# Autodesk Inventor assembly: ASY МОО 001 отстойник осветлитель
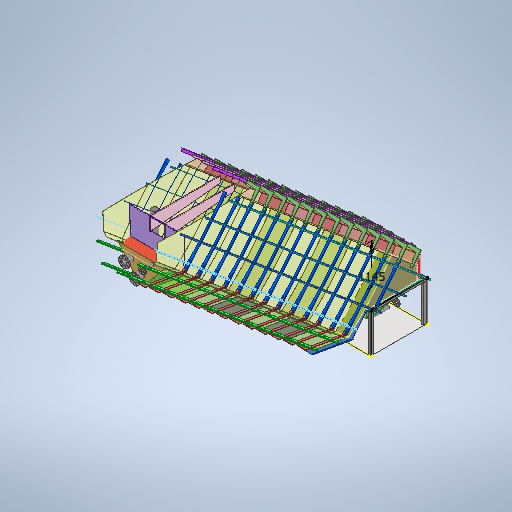
[picture p0: Inventor's stored thumbnail of the model, 512x512]
Saved by Autodesk Inventor 2025 (Build 290162010, 162A)
## iProperties
Created: 2024-04-28
Part Number: ASY МОО 001 отстойник осветлитель
Document SubType Name: Weldment
Designer: admin
Weld Material: Welded Aluminum-6061
Mass: 1.58517e+06 g
Surface Area: 1.48953e+06 cm^2
Volume: 226523 cm^3
Density: 6.99781 g/cm^3
Author: admin
## Documents named in this file (51)
- C:\Users\admin\YandexDisk-badmisterfox\домашниий пк\Inventor\Manturovo\Manturovo_Se-clar\ASY МОО 001 отстойник осветлитель.iam
- C:\Users\admin\YandexDisk-badmisterfox\домашниий пк\Inventor\Manturovo\Manturovo_Se-clar\MSC 033 sheet back basic.ipt
- C:\Users\admin\YandexDisk-badmisterfox\домашниий пк\Inventor\Manturovo\Manturovo_Se-clar\Пример емкости.ipt
- C:\Users\admin\YandexDisk-badmisterfox\домашниий пк\Inventor\Manturovo\Manturovo_Se-clar\MSC 041 sheet belly main.ipt
- C:\Users\admin\YandexDisk-badmisterfox\домашниий пк\Inventor\Manturovo\Manturovo_Se-clar\MSC 052 rib board.ipt
- C:\Users\admin\YandexDisk-badmisterfox\домашниий пк\Inventor\Manturovo\Manturovo_Se-clar\MSC 051 rib back.ipt
- C:\Users\admin\YandexDisk-badmisterfox\домашниий пк\Inventor\Manturovo\Manturovo_Se-clar\Рама основания\ASY MSC 090 base frame.iam
- C:\Users\admin\YandexDisk-badmisterfox\домашниий пк\Inventor\Manturovo\Manturovo_Se-clar\ASY MSC 080 roсket.iam
- C:\Users\admin\YandexDisk-badmisterfox\домашниий пк\Inventor\Manturovo\Manturovo_Se-clar\Content Center Files\en-US\ISO 5251 B 3D\ISO 5251 Bends 3D without straight ends(90 deg) DN80 2 2.ipt
- C:\Users\admin\YandexDisk-badmisterfox\домашниий пк\Inventor\Manturovo\Manturovo_Se-clar\Content Center Files\en-US\ISO 5251(1)\ISO 5251 Concentric reducers DN80 x DN65 3,2 3,2.ipt
- C:\Users\admin\YandexDisk-badmisterfox\домашниий пк\Inventor\Manturovo\Manturovo_Se-clar\ASY MSC 010 cone.iam
- C:\Users\admin\YandexDisk-badmisterfox\домашниий пк\Inventor\Manturovo\Manturovo_Se-clar\ракета\МОО 064 ракета труба.ipt
- C:\Users\admin\YandexDisk-badmisterfox\домашниий пк\Inventor\Manturovo\Manturovo_Se-clar\MSC 000 DIM settler-clarifier.ipt
- C:\Users\admin\YandexDisk-badmisterfox\домашниий пк\Inventor\Manturovo\Manturovo_Se-clar\MSC 031 sheet lowerback.ipt
- C:\Users\admin\YandexDisk-badmisterfox\домашниий пк\Inventor\Manturovo\Manturovo_Se-clar\Content Center Files\en-US\DIN EN 1092-1 01 - PN 25\DIN EN 1092-1 Plate Flange for Welding Type 01 - PN 25 80 x 88.9.ipt
- C:\Users\admin\YandexDisk-badmisterfox\домашниий пк\Inventor\Manturovo\Manturovo_Se-clar\MSC 024 sheet board main.ipt
- C:\Users\admin\YandexDisk-badmisterfox\домашниий пк\Inventor\Manturovo\Manturovo_Se-clar\MSC 032 sheet magic back-lowerback.ipt
- C:\Users\admin\YandexDisk-badmisterfox\домашниий пк\Inventor\Manturovo\Manturovo_Se-clar\MSC 021 sheet left board hip.ipt
- C:\Users\admin\YandexDisk-badmisterfox\домашниий пк\Inventor\Manturovo\Manturovo_Se-clar\MSC 022 sheet right board hip.ipt
- C:\Users\admin\YandexDisk-badmisterfox\домашниий пк\Inventor\Manturovo\Manturovo_Se-clar\MSC 034 sheet back-neck.ipt
- C:\Users\admin\YandexDisk-badmisterfox\домашниий пк\Inventor\Manturovo\Manturovo_Se-clar\MSC 042 sheet belly-neck.ipt
- C:\Users\admin\YandexDisk-badmisterfox\домашниий пк\Inventor\Manturovo\Manturovo_Se-clar\MSC 023 sheet board.ipt
- C:\Users\admin\YandexDisk-badmisterfox\домашниий пк\Inventor\Manturovo\Manturovo_Se-clar\конус\MSC 071 ridge 1.ipt
- C:\Users\admin\YandexDisk-badmisterfox\домашниий пк\Inventor\Manturovo\Manturovo_Se-clar\конус\MSC 073 ridge 3.ipt
- C:\Users\admin\YandexDisk-badmisterfox\домашниий пк\Inventor\Manturovo\Manturovo_Se-clar\конус\MSC 074 face 1.ipt
- C:\Users\admin\YandexDisk-badmisterfox\домашниий пк\Inventor\Manturovo\Manturovo_Se-clar\Content Center Files\en-US\ISO 5251 B 3D\ISO 5251 Bends 3D without straight ends(90 deg) DN150 11 11.ipt
- C:\Users\admin\YandexDisk-badmisterfox\домашниий пк\Inventor\Manturovo\Manturovo_Se-clar\Content Center Files\en-US\DIN EN 1092-1 01 - PN 25\DIN EN 1092-1 Plate Flange for Welding Type 01 - PN 25 150 x 168.3.ipt
- C:\Users\admin\YandexDisk-badmisterfox\домашниий пк\Inventor\Manturovo\Manturovo_Se-clar\МОО 061 труба верх 1.ipt
- C:\Users\admin\YandexDisk-badmisterfox\домашниий пк\Inventor\Manturovo\Manturovo_Se-clar\МОО 062 труба верх 2.ipt
- C:\Users\admin\YandexDisk-badmisterfox\домашниий пк\Inventor\Manturovo\Manturovo_Se-clar\МОО 063 труба верх 3.ipt
- C:\Users\admin\YandexDisk-badmisterfox\домашниий пк\Inventor\Manturovo\Manturovo_Se-clar\MSC 061 stringer back ^.ipt
- C:\Users\admin\YandexDisk-badmisterfox\домашниий пк\Inventor\Manturovo\Manturovo_Se-clar\MSC 063 stringer board #.ipt
- C:\Users\admin\YandexDisk-badmisterfox\домашниий пк\Inventor\Manturovo\Manturovo_Se-clar\MSC 062 stringer back ^^.ipt
- C:\Users\admin\YandexDisk-badmisterfox\домашниий пк\Inventor\Manturovo\Manturovo_Se-clar\MSC 064 stringer board ##.ipt
- C:\Users\admin\YandexDisk-badmisterfox\домашниий пк\Inventor\Manturovo\Manturovo_Se-clar\MSC 065 stringer board ###.ipt
- C:\Users\admin\YandexDisk-badmisterfox\домашниий пк\Inventor\Manturovo\Manturovo_Se-clar\MSC 066 stringer board ####.ipt
- C:\Users\admin\YandexDisk-badmisterfox\домашниий пк\Inventor\Manturovo\Manturovo_Se-clar\MSC 067 stringer board belly.ipt
- C:\Users\admin\YandexDisk-badmisterfox\домашниий пк\Inventor\Manturovo\Manturovo_Se-clar\MSC 053 rib belly.ipt
- C:\Users\admin\YandexDisk-badmisterfox\домашниий пк\Inventor\Manturovo\Manturovo_Se-clar\MSC 025 sheet board withers 1.ipt
- C:\Users\admin\YandexDisk-badmisterfox\домашниий пк\Inventor\Manturovo\Manturovo_Se-clar\MSC 027 sheet board face 1.ipt
- C:\Users\admin\YandexDisk-badmisterfox\домашниий пк\Inventor\Manturovo\Manturovo_Se-clar\Part1.ipt
- C:\Users\admin\YandexDisk-badmisterfox\домашниий пк\Inventor\Manturovo\Manturovo_Se-clar\стапель\ASY стапель.iam
- C:\Users\admin\YandexDisk-badmisterfox\домашниий пк\Inventor\Manturovo\Manturovo_Se-clar\DXF файлы\Шпангоуты+стрингеры\MSC 0101 sheet gills.ipt
- C:\Users\admin\YandexDisk-badmisterfox\домашниий пк\Inventor\Manturovo\Manturovo_Se-clar\MSC 026 sheet board withers 2.ipt
- C:\Users\admin\YandexDisk-badmisterfox\домашниий пк\Inventor\Manturovo\Manturovo_Se-clar\MSC 028 sheet board face 2.ipt
- C:\Users\admin\YandexDisk-badmisterfox\домашниий пк\Inventor\Manturovo\Manturovo_Se-clar\MSC 068 stringer lowerback.ipt
- C:\Users\admin\YandexDisk-badmisterfox\домашниий пк\Inventor\Manturovo\Manturovo_Se-clar\конус\MSC 072 ridge 2.ipt
- C:\Users\admin\YandexDisk-badmisterfox\домашниий пк\Inventor\Manturovo\Manturovo_Se-clar\MSC 075 face 2.ipt
- C:\Users\admin\YandexDisk-badmisterfox\домашниий пк\Inventor\Manturovo\Manturovo_Se-clar\MSC 076 face 3.ipt
- C:\Users\admin\YandexDisk-badmisterfox\домашниий пк\Inventor\Manturovo\Manturovo_Se-clar\MSC 077 face 4.ipt
- C:\Users\admin\YandexDisk-badmisterfox\домашниий пк\Inventor\Manturovo\Manturovo_Se-clar\MSC 052 rib board_CPY.ipt
## Components (226 placed, 57 different names)
1. Пример емкости.ipt:1 — Mate:1, Mate:2, Flush:2
2. MSC 000 DIM settler-clarifier.ipt:1
3. ASY MSC 090 base frame.iam:1 [sub-assembly] — Flush:19, Flush:21, Mate:82
4. MSC 033 sheet back basic.ipt:1 — Flush:3, Rigid:11, Rigid:12
5. MSC 041 sheet belly main.ipt:1 — Mate:9, Rigid:18, Rigid:40
6. ASY MSC 080 roсket.iam:1 [sub-assembly] — Flush:23, Rigid:10
7. ISO 5251 Bends 3D without straight ends(90 deg) DN80 2 2.ipt:1 — Rigid:2, Rigid:3
8. ISO 5251 Concentric reducers DN80 x DN65 3,2 3,2.ipt:1 — Rigid:2, Rigid:10, Mate:79
9. ASY MSC 010 cone.iam:1 [sub-assembly] — Flush:22, Mate:16, Flush:28, Mate:31, Mate:36, Mate:54, Mate:57, Mate:65, Mate:78, Tangent:11, Mate:79, Flush:79, Mate:82
10. МОО 064 ракета труба.ipt:1 — Rigid:3, Cylindrical:1
11. MSC 033 sheet back basic.ipt:2 — Rigid:11, Tangent:1, Tangent:3, Rigid:37
12. MSC 033 sheet back basic.ipt:3 — Flush:24, Rigid:12, Mate:19, Mate:22, Rigid:30, Mate:31, Flush:44, Tangent:8, Tangent:9
13. MSC 031 sheet lowerback.ipt:1 — Mate:15, Mate:16, Mate:19, Mate:22, Tangent:10, Tangent:11
14. DIN EN 1092-1 Plate Flange for Welding Type 01 - PN 25 80 x 88.9.ipt:1 — Flush:25, Flush:26, Mate:18, Cylindrical:1
15. MSC 024 sheet board main.ipt:1 — Flush:30, Tangent:1, Rigid:35, Mate:37
16. MSC 041 sheet belly main.ipt:2 — Rigid:18, Rigid:53
17. MSC 032 sheet magic back-lowerback.ipt:1 — Mate:24, Rigid:30, Flush:42, Tangent:6, Flush:43, Tangent:7
18. MSC 021 sheet left board hip.ipt:1 — Flush:41, Flush:42, Tangent:6, Mate:78
19. MSC 022 sheet right board hip.ipt:1 — Mate:30, Flush:43, Tangent:7
20. MSC 024 sheet board main.ipt:2 — Rigid:35, Rigid:36
21. MSC 024 sheet board main.ipt:3 — Rigid:36, Rigid:49
22. MSC 033 sheet back basic.ipt:4 — Rigid:37, Rigid:38
23. MSC 033 sheet back basic.ipt:5 — Rigid:38, Rigid:39
24. MSC 034 sheet back-neck.ipt:1 — Rigid:39
25. MSC 041 sheet belly main.ipt:3 — Rigid:40, Rigid:47
26. MSC 042 sheet belly-neck.ipt:1 — Rigid:48, Mate:70, Mate:71
27. MSC 041 sheet belly main.ipt:4 — Rigid:45, Rigid:47
28. MSC 041 sheet belly main.ipt:5 — Rigid:45, Rigid:48
29. MSC 024 sheet board main.ipt:4 — Rigid:49, Rigid:50
30. MSC 024 sheet board main.ipt:5 — Rigid:50, Rigid:113
31. MSC 023 sheet board.ipt:1 — Mate:36, Flush:47, Tangent:8, Mate:37, Mate:55
32. MSC 071 ridge 1.ipt:1 — Mate:50, Flush:57, Mate:68, Flush:81
33. MSC 074 face 1.ipt:1 — Rigid:156, Rigid:157, Mate:70, Flush:62, Mate:71, Rigid:159, Mate:80
34. MSC 041 sheet belly main.ipt:6 — Mate:54, Mate:55, Rigid:53
35. DIN EN 1092-1 Plate Flange for Welding Type 01 - PN 25 80 x 88.9.ipt:2 — Rigid:62
36. MSC 073 ridge 3.ipt:1 — Flush:56, Flush:57, Mate:68, Mate:77, Flush:78, Mate:81, Flush:80
37. DIN EN 1092-1 Plate Flange for Welding Type 01 - PN 25 150 x 168.3.ipt:1 — Rigid:158
38. МОО 061 труба верх 1.ipt:1 — Rigid:158, Rigid:59, Rigid:159
39. ISO 5251 Bends 3D without straight ends(90 deg) DN150 11 11.ipt:1 — Rigid:59, Rotational:2
40. МОО 062 труба верх 2.ipt:1 — Rigid:132, Rigid:156
41. DIN EN 1092-1 Plate Flange for Welding Type 01 - PN 25 150 x 168.3.ipt:2 — Rigid:132
42. МОО 063 труба верх 3.ipt:1 — Rigid:62, Rigid:157
43. MSC 024 sheet board main.ipt:6 — Rigid:134
44. MSC 024 sheet board main.ipt:7
45. MSC 024 sheet board main.ipt:8
46. MSC 024 sheet board main.ipt:9
47. MSC 024 sheet board main.ipt:10 — Rigid:67
48. MSC 023 sheet board.ipt:2 — Rigid:67, Mate:57, Mate:58, Tangent:9
49. MSC 052 rib board.ipt:1 — Rigid:74, Rigid:161, Rigid:162, Rigid:163, Rigid:164
50. MSC 051 rib back.ipt:1 — Rigid:25, Rigid:74, Rigid:91, Rigid:93, Rigid:139
51. MSC 066 stringer board ####.ipt:1 — Rigid:143, Rigid:162
52. MSC 065 stringer board ###.ipt:1 — Rigid:142, Rigid:163
53. MSC 064 stringer board ##.ipt:1 — Rigid:141, Rigid:164
54. MSC 063 stringer board #.ipt:1 — Rigid:140
55. MSC 062 stringer back ^^.ipt:1 — Rigid:93, Rigid:155
56. MSC 061 stringer back ^.ipt:2 — Rigid:91, Rigid:153
57. MSC 061 stringer back ^.ipt:1 — Rigid:90, Rigid:152
58. MSC 025 sheet board withers 1.ipt:1 — Rigid:113, Rigid:114
59. MSC 027 sheet board face 1.ipt:1 — Rigid:114, Flush:56, Mate:69, Flush:60, Mate:75
60. Part1.ipt:1
61. MSC 051 rib back.ipt:2 — Rigid:116, Rigid:130, Rigid:131, Rigid:169
62. MSC 051 rib back.ipt:3 — Rigid:116, Rigid:165
63. MSC 051 rib back.ipt:4 — Rigid:131
64. MSC 051 rib back.ipt:5 — Mate:62, Flush:53
65. MSC 062 stringer back ^^.ipt:2 — Rigid:92, Mate:66, Rigid:154
66. MSC 066 stringer board ####.ipt:2 — Rigid:125, Rigid:151
67. MSC 063 stringer board #.ipt:2 — Rigid:148
68. MSC 064 stringer board ##.ipt:2 — Rigid:149, Rigid:167
69. MSC 065 stringer board ###.ipt:2 — Rigid:150, Rigid:166
70. MSC 052 rib board.ipt:3 — Rigid:72, Flush:51, Flush:52, Rigid:125, Mate:61, Rigid:166, Rigid:167, Rigid:168
71. MSC 051 rib back.ipt:6 — Flush:12, Tangent:3, Rigid:25, Flush:44, Rigid:72, Rigid:90, Rigid:92, Rigid:130
72. ASY стапель.iam:1 [sub-assembly] — Mate:62, Flush:53, Mate:63
73. MSC 053 rib belly.ipt:2 — Rigid:110, Flush:51, Flush:52, Rigid:126, Mate:61, Rigid:127
74. MSC 053 rib belly.ipt:1 — Rigid:111, Rigid:112, Rigid:127
75. MSC 067 stringer board belly.ipt:4 — Rigid:126, Rigid:147
76. MSC 067 stringer board belly.ipt:3 — Rigid:110, Rigid:146
77. MSC 067 stringer board belly.ipt:2 — Rigid:112, Rigid:144
78. MSC 067 stringer board belly.ipt:1 — Rigid:111, Rigid:145
79. MSC 0101 sheet gills.ipt:1 — Mate:64
80. MSC 026 sheet board withers 2.ipt:1 — Rigid:133, Rigid:134
81. MSC 028 sheet board face 2.ipt:1 — Rigid:133
82. MSC 068 stringer lowerback.ipt:1 — Mate:65, Mate:66, Tangent:10
83. MSC 072 ridge 2.ipt:1 — Flush:58, Mate:81, Flush:80, Flush:81
84. МОО 061 труба верх 1.ipt:2 — Rotational:2
85. MSC 075 face 2.ipt:1 — Mate:69, Flush:60, Flush:61, Mate:76
86. MSC 076 face 3.ipt:1 — Flush:76, Mate:75, Mate:76
87. MSC 077 face 4.ipt:1 — Mate:77, Flush:77, Flush:78, Mate:80
88. MSC 066 stringer board ####.ipt:9 — Rigid:160
89. MSC 052 rib board_CPY:1 — Rigid:169
90. MSC 052 rib board_CPY:2 — Rigid:165
91. MSC 053 rib belly.ipt:3
92. MSC 052 rib board.ipt:4
93. MSC 051 rib back.ipt:7 — Rigid:139
94. MSC 051 rib back.ipt:8
95. MSC 052 rib board.ipt:5
96. MSC 053 rib belly.ipt:4
97. MSC 053 rib belly.ipt:5
98. MSC 052 rib board.ipt:6
99. MSC 051 rib back.ipt:9
100. MSC 051 rib back.ipt:10
101. MSC 052 rib board.ipt:7
102. MSC 053 rib belly.ipt:6
103. MSC 053 rib belly.ipt:7
104. MSC 052 rib board.ipt:8
105. MSC 051 rib back.ipt:11
106. MSC 051 rib back.ipt:12
107. MSC 052 rib board.ipt:9
108. MSC 053 rib belly.ipt:8
109. MSC 053 rib belly.ipt:9
110. MSC 052 rib board.ipt:10
111. MSC 051 rib back.ipt:13
112. MSC 051 rib back.ipt:14
113. MSC 052 rib board.ipt:11
114. MSC 053 rib belly.ipt:10
115. MSC 053 rib belly.ipt:11
116. MSC 052 rib board.ipt:12
117. MSC 051 rib back.ipt:15
118. MSC 051 rib back.ipt:16
119. MSC 052 rib board.ipt:13
120. MSC 053 rib belly.ipt:12
121. MSC 053 rib belly.ipt:13
122. MSC 052 rib board.ipt:14
123. MSC 051 rib back.ipt:17
124. MSC 051 rib back.ipt:18
125. MSC 052 rib board.ipt:15
126. MSC 053 rib belly.ipt:14
127. MSC 053 rib belly.ipt:15
128. MSC 052 rib board.ipt:16
129. MSC 051 rib back.ipt:19
130. MSC 051 rib back.ipt:20
131. MSC 052 rib board.ipt:17
132. MSC 053 rib belly.ipt:16
133. MSC 053 rib belly.ipt:17
134. MSC 052 rib board.ipt:18
135. MSC 051 rib back.ipt:21
136. MSC 051 rib back.ipt:22
137. MSC 052 rib board.ipt:19
138. MSC 053 rib belly.ipt:18
139. MSC 053 rib belly.ipt:19
140. MSC 052 rib board.ipt:20
141. MSC 051 rib back.ipt:23
142. MSC 051 rib back.ipt:24
143. MSC 052 rib board.ipt:21
144. MSC 053 rib belly.ipt:20
145. MSC 053 rib belly.ipt:21
146. MSC 052 rib board.ipt:22
147. MSC 051 rib back.ipt:25
148. MSC 051 rib back.ipt:26
149. MSC 052 rib board.ipt:23
150. MSC 053 rib belly.ipt:22
151. MSC 053 rib belly.ipt:23
152. MSC 052 rib board.ipt:24
153. MSC 051 rib back.ipt:27
154. MSC 051 rib back.ipt:28
155. MSC 052 rib board.ipt:25
156. MSC 053 rib belly.ipt:24
157. MSC 053 rib belly.ipt:25
158. MSC 052 rib board.ipt:26
159. MSC 051 rib back.ipt:29
160. MSC 051 rib back.ipt:30
161. MSC 052 rib board.ipt:27
162. MSC 053 rib belly.ipt:26
163. MSC 063 stringer board #.ipt:3 — Rigid:148, Rigid:168
164. MSC 064 stringer board ##.ipt:3 — Rigid:149
165. MSC 065 stringer board ###.ipt:3 — Rigid:150
166. MSC 066 stringer board ####.ipt:3 — Rigid:151
167. MSC 067 stringer board belly.ipt:5 — Rigid:147
168. MSC 067 stringer board belly.ipt:6 — Rigid:146
169. MSC 062 stringer back ^^.ipt:3 — Rigid:154
170. MSC 061 stringer back ^.ipt:3 — Rigid:152
171. MSC 061 stringer back ^.ipt:4 — Rigid:153
172. MSC 062 stringer back ^^.ipt:4 — Rigid:155
173. MSC 063 stringer board #.ipt:4 — Rigid:140, Rigid:161
174. MSC 064 stringer board ##.ipt:4 — Rigid:141
175. MSC 065 stringer board ###.ipt:4 — Rigid:142
176. MSC 066 stringer board ####.ipt:4 — Rigid:143
177. MSC 067 stringer board belly.ipt:7 — Rigid:145
178. MSC 067 stringer board belly.ipt:8 — Rigid:144
179. MSC 063 stringer board #.ipt:5
180. MSC 064 stringer board ##.ipt:5
181. MSC 065 stringer board ###.ipt:5
182. MSC 066 stringer board ####.ipt:5
183. MSC 067 stringer board belly.ipt:9
184. MSC 067 stringer board belly.ipt:10
185. MSC 062 stringer back ^^.ipt:5
186. MSC 061 stringer back ^.ipt:5
187. MSC 061 stringer back ^.ipt:6
188. MSC 062 stringer back ^^.ipt:6
189. MSC 063 stringer board #.ipt:6
190. MSC 064 stringer board ##.ipt:6
191. MSC 065 stringer board ###.ipt:6
192. MSC 066 stringer board ####.ipt:6
193. MSC 067 stringer board belly.ipt:11
194. MSC 067 stringer board belly.ipt:12
195. MSC 063 stringer board #.ipt:7
196. MSC 064 stringer board ##.ipt:7
197. MSC 065 stringer board ###.ipt:7
198. MSC 066 stringer board ####.ipt:7
199. MSC 067 stringer board belly.ipt:13
200. MSC 067 stringer board belly.ipt:14
201. MSC 062 stringer back ^^.ipt:7
202. MSC 061 stringer back ^.ipt:7
203. MSC 061 stringer back ^.ipt:8
204. MSC 062 stringer back ^^.ipt:8
205. MSC 063 stringer board #.ipt:8
206. MSC 064 stringer board ##.ipt:8
207. MSC 065 stringer board ###.ipt:8
208. MSC 066 stringer board ####.ipt:8 — Rigid:160
209. MSC 067 stringer board belly.ipt:15
210. MSC 067 stringer board belly.ipt:16
211. МОО 053 стрингер борт 3:9
212. МОО 054 стрингер борт 4:9
213. МОО 055 стрингер борт 5:9
214. МОО 056 стрингер борт 6:10
215. МОО 057 стрингер борт 7:19
216. МОО 057 стрингер борт 7:20
217. МОО 052 стрингер спина 2:9
218. МОО 051 стрингер спина 1:9
219. МОО 051 стрингер спина 1:10
220. МОО 052 стрингер спина 2:10
221. МОО 053 стрингер борт 3:10
222. МОО 054 стрингер борт 4:10
223. МОО 055 стрингер борт 5:10
224. МОО 056 стрингер борт 6:11
225. МОО 057 стрингер борт 7:21
226. МОО 057 стрингер борт 7:22
## Component patterns: (12 elements, first: MSC 053 rib belly.ipt:3 + MSC 052 rib board.ipt:4 + MSC 051 rib back.ipt:7 + MSC 051 rib back.ipt:8 + MSC 052 rib board.ipt:5 + MSC 053 rib belly.ipt:4), (4 elements, first: MSC 063 stringer board #.ipt:3 + MSC 064 stringer board ##.ipt:3 + MSC 065 stringer board ###.ipt:3 + MSC 066 stringer board ####.ipt:3 + MSC 067 stringer board belly.ipt:5 + MSC 067 stringer board belly.ipt:6 + MSC 062 stringer back ^^.ipt:3 + MSC 061 stringer back ^.ipt:3 + MSC 061 stringer back ^.ipt:4 + MSC 062 stringer back ^^.ipt:4 + MSC 063 stringer board #.ipt:4 + MSC 064 stringer board ##.ipt:4 + MSC 065 stringer board ###.ipt:4 + MSC 066 stringer board ####.ipt:4 + MSC 067 stringer board belly.ipt:7 + MSC 067 stringer board belly.ipt:8)
## Relationships (164: WeldJoint 83, Mate 37, Flush 34, Tangent 8, CylindricalJoint 1, RevoluteJoint 1)
- Mate:1: Пример емкости.ipt:1
- Mate:2: Пример емкости.ipt:1
- Flush:2: Пример емкости.ipt:1
- Flush:3: MSC 033 sheet back basic.ipt:1
- Mate:9: MSC 041 sheet belly main.ipt:1
- Flush:12: MSC 051 rib back.ipt:6
- Rigid:2 [WeldJoint]: ISO 5251 Bends 3D without straight ends(90 deg) DN80 2 2.ipt:1 ↔ ISO 5251 Concentric reducers DN80 x DN65 3,2 3,2.ipt:1
- Rigid:3 [WeldJoint]: ISO 5251 Bends 3D without straight ends(90 deg) DN80 2 2.ipt:1 ↔ МОО 064 ракета труба.ipt:1
- Flush:19: ASY MSC 090 base frame.iam:1
- Flush:21: ASY MSC 090 base frame.iam:1
- Flush:22: ASY MSC 010 cone.iam:1
- Flush:23: ASY MSC 080 roсket.iam:1
- Mate:15: MSC 031 sheet lowerback.ipt:1
- Flush:24: MSC 033 sheet back basic.ipt:3
- Mate:16: ASY MSC 010 cone.iam:1 ↔ MSC 031 sheet lowerback.ipt:1
- Flush:25: DIN EN 1092-1 Plate Flange for Welding Type 01 - PN 25 80 x 88.9.ipt:1
- Flush:26: DIN EN 1092-1 Plate Flange for Welding Type 01 - PN 25 80 x 88.9.ipt:1
- Mate:18 (120 mm): DIN EN 1092-1 Plate Flange for Welding Type 01 - PN 25 80 x 88.9.ipt:1
- Rigid:10 [WeldJoint] (-20 mm): ASY MSC 080 roсket.iam:1 ↔ ISO 5251 Concentric reducers DN80 x DN65 3,2 3,2.ipt:1
- Cylindrical:1: МОО 064 ракета труба.ipt:1 ↔ DIN EN 1092-1 Plate Flange for Welding Type 01 - PN 25 80 x 88.9.ipt:1
- Flush:28: ASY MSC 010 cone.iam:1
- Rigid:11 [WeldJoint]: MSC 033 sheet back basic.ipt:1 ↔ MSC 033 sheet back basic.ipt:2
- Rigid:12 [WeldJoint]: MSC 033 sheet back basic.ipt:1 ↔ MSC 033 sheet back basic.ipt:3
- Mate:19 (910 mm): MSC 033 sheet back basic.ipt:3 ↔ MSC 031 sheet lowerback.ipt:1
- Flush:30: MSC 024 sheet board main.ipt:1
- Tangent:1: MSC 033 sheet back basic.ipt:2 ↔ MSC 024 sheet board main.ipt:1
- Tangent:3: MSC 033 sheet back basic.ipt:2 ↔ MSC 051 rib back.ipt:6
- Mate:22 (47 mm): MSC 033 sheet back basic.ipt:3 ↔ MSC 031 sheet lowerback.ipt:1
- Rigid:18 [WeldJoint]: MSC 041 sheet belly main.ipt:1 ↔ MSC 041 sheet belly main.ipt:2
- Rigid:25 [WeldJoint] (-50 mm): MSC 051 rib back.ipt:1 ↔ MSC 051 rib back.ipt:6
- Mate:24: MSC 032 sheet magic back-lowerback.ipt:1
- Rigid:30 [WeldJoint]: MSC 033 sheet back basic.ipt:3 ↔ MSC 032 sheet magic back-lowerback.ipt:1
- Flush:41: MSC 021 sheet left board hip.ipt:1
- Flush:42: MSC 032 sheet magic back-lowerback.ipt:1 ↔ MSC 021 sheet left board hip.ipt:1
- Tangent:6: MSC 032 sheet magic back-lowerback.ipt:1 ↔ MSC 021 sheet left board hip.ipt:1
- Mate:30: MSC 022 sheet right board hip.ipt:1
- Flush:43: MSC 032 sheet magic back-lowerback.ipt:1 ↔ MSC 022 sheet right board hip.ipt:1
- Tangent:7: MSC 032 sheet magic back-lowerback.ipt:1 ↔ MSC 022 sheet right board hip.ipt:1
- Rigid:35 [WeldJoint]: MSC 024 sheet board main.ipt:1 ↔ MSC 024 sheet board main.ipt:2
- Rigid:36 [WeldJoint]: MSC 024 sheet board main.ipt:2 ↔ MSC 024 sheet board main.ipt:3
- Rigid:37 [WeldJoint]: MSC 033 sheet back basic.ipt:2 ↔ MSC 033 sheet back basic.ipt:4
- Rigid:38 [WeldJoint]: MSC 033 sheet back basic.ipt:4 ↔ MSC 033 sheet back basic.ipt:5
- Rigid:39 [WeldJoint]: MSC 033 sheet back basic.ipt:5 ↔ MSC 034 sheet back-neck.ipt:1
- Mate:31: ASY MSC 010 cone.iam:1 ↔ MSC 033 sheet back basic.ipt:3
- Rigid:40 [WeldJoint]: MSC 041 sheet belly main.ipt:1 ↔ MSC 041 sheet belly main.ipt:3
- Flush:44 (-250 mm): MSC 033 sheet back basic.ipt:3 ↔ MSC 051 rib back.ipt:6
- Rigid:45 [WeldJoint]: MSC 041 sheet belly main.ipt:4 ↔ MSC 041 sheet belly main.ipt:5
- Rigid:47 [WeldJoint]: MSC 041 sheet belly main.ipt:3 ↔ MSC 041 sheet belly main.ipt:4
- Rigid:48 [WeldJoint]: MSC 042 sheet belly-neck.ipt:1 ↔ MSC 041 sheet belly main.ipt:5
- Rigid:49 [WeldJoint]: MSC 024 sheet board main.ipt:3 ↔ MSC 024 sheet board main.ipt:4
- Rigid:50 [WeldJoint]: MSC 024 sheet board main.ipt:4 ↔ MSC 024 sheet board main.ipt:5
- Mate:36: ASY MSC 010 cone.iam:1 ↔ MSC 023 sheet board.ipt:1
- Flush:47: MSC 023 sheet board.ipt:1
- Tangent:8: MSC 033 sheet back basic.ipt:3 ↔ MSC 023 sheet board.ipt:1
- Mate:37: MSC 024 sheet board main.ipt:1 ↔ MSC 023 sheet board.ipt:1
- Mate:50 (200 mm): MSC 071 ridge 1.ipt:1
- Mate:54: ASY MSC 010 cone.iam:1 ↔ MSC 041 sheet belly main.ipt:6
- Mate:55: MSC 023 sheet board.ipt:1 ↔ MSC 041 sheet belly main.ipt:6
- Rigid:53 [WeldJoint]: MSC 041 sheet belly main.ipt:2 ↔ MSC 041 sheet belly main.ipt:6
- Rigid:158 [WeldJoint]: DIN EN 1092-1 Plate Flange for Welding Type 01 - PN 25 150 x 168.3.ipt:1 ↔ МОО 061 труба верх 1.ipt:1
- Rigid:59 [WeldJoint]: МОО 061 труба верх 1.ipt:1 ↔ ISO 5251 Bends 3D without straight ends(90 deg) DN150 11 11.ipt:1
- Rigid:62 [WeldJoint]: DIN EN 1092-1 Plate Flange for Welding Type 01 - PN 25 80 x 88.9.ipt:2 ↔ МОО 063 труба верх 3.ipt:1
- [WeldJoint]: MSC 024 sheet board main.ipt:6 ↔ MSC 024 sheet board main.ipt:7
- [WeldJoint]: MSC 024 sheet board main.ipt:7 ↔ MSC 024 sheet board main.ipt:8
- [WeldJoint]: MSC 024 sheet board main.ipt:8 ↔ MSC 024 sheet board main.ipt:9
- [WeldJoint]: MSC 024 sheet board main.ipt:9 ↔ MSC 024 sheet board main.ipt:10
- Rigid:67 [WeldJoint]: MSC 024 sheet board main.ipt:10 ↔ MSC 023 sheet board.ipt:2
- Mate:57: ASY MSC 010 cone.iam:1 ↔ MSC 023 sheet board.ipt:2
- Mate:58: MSC 023 sheet board.ipt:2
- Tangent:9: MSC 033 sheet back basic.ipt:3 ↔ MSC 023 sheet board.ipt:2
- Rigid:72 [WeldJoint] (-50 mm): MSC 052 rib board.ipt:3 ↔ MSC 051 rib back.ipt:6
- Rigid:74 [WeldJoint] (-50 mm): MSC 052 rib board.ipt:1 ↔ MSC 051 rib back.ipt:1
- Rigid:90 [WeldJoint] (2 mm): MSC 061 stringer back ^.ipt:1 ↔ MSC 051 rib back.ipt:6
- Rigid:91 [WeldJoint] (2 mm): MSC 051 rib back.ipt:1 ↔ MSC 061 stringer back ^.ipt:2
- Rigid:92 [WeldJoint] (2 mm): MSC 062 stringer back ^^.ipt:2 ↔ MSC 051 rib back.ipt:6
- Rigid:93 [WeldJoint] (2 mm): MSC 051 rib back.ipt:1 ↔ MSC 062 stringer back ^^.ipt:1
- Rigid:110 [WeldJoint] (2 mm): MSC 053 rib belly.ipt:2 ↔ MSC 067 stringer board belly.ipt:3
- Rigid:111 [WeldJoint] (2 mm): MSC 053 rib belly.ipt:1 ↔ MSC 067 stringer board belly.ipt:1
- Rigid:112 [WeldJoint] (2 mm): MSC 053 rib belly.ipt:1 ↔ MSC 067 stringer board belly.ipt:2
- Rigid:113 [WeldJoint]: MSC 024 sheet board main.ipt:5 ↔ MSC 025 sheet board withers 1.ipt:1
- Rigid:114 [WeldJoint]: MSC 025 sheet board withers 1.ipt:1 ↔ MSC 027 sheet board face 1.ipt:1
- Rigid:116 [WeldJoint] (50 mm): MSC 051 rib back.ipt:2 ↔ MSC 051 rib back.ipt:3
- [WeldJoint] (50 mm): MSC 051 rib back.ipt:4 ↔ MSC 051 rib back.ipt:5
- Flush:51: MSC 052 rib board.ipt:3 ↔ MSC 053 rib belly.ipt:2
- Flush:52: MSC 052 rib board.ipt:3 ↔ MSC 053 rib belly.ipt:2
- Rigid:125 [WeldJoint] (2 mm): MSC 066 stringer board ####.ipt:2 ↔ MSC 052 rib board.ipt:3
- Rigid:126 [WeldJoint] (2 mm): MSC 053 rib belly.ipt:2 ↔ MSC 067 stringer board belly.ipt:4
- Mate:61: MSC 052 rib board.ipt:3 ↔ MSC 053 rib belly.ipt:2
- Mate:62: MSC 051 rib back.ipt:5 ↔ ASY стапель.iam:1
- Flush:53: MSC 051 rib back.ipt:5 ↔ ASY стапель.iam:1
- Mate:63: ASY стапель.iam:1
- Rigid:127 [WeldJoint] (-50 mm): MSC 053 rib belly.ipt:2 ↔ MSC 053 rib belly.ipt:1
- Rigid:130 [WeldJoint] (-500 mm): MSC 051 rib back.ipt:2 ↔ MSC 051 rib back.ipt:6
- Rigid:131 [WeldJoint] (-500 mm): MSC 051 rib back.ipt:2 ↔ MSC 051 rib back.ipt:4
- Rigid:132 [WeldJoint]: МОО 062 труба верх 2.ipt:1 ↔ DIN EN 1092-1 Plate Flange for Welding Type 01 - PN 25 150 x 168.3.ipt:2
- Mate:64: MSC 0101 sheet gills.ipt:1
- Rigid:133 [WeldJoint]: MSC 026 sheet board withers 2.ipt:1 ↔ MSC 028 sheet board face 2.ipt:1
- Rigid:134 [WeldJoint]: MSC 024 sheet board main.ipt:6 ↔ MSC 026 sheet board withers 2.ipt:1
- Mate:65: ASY MSC 010 cone.iam:1 ↔ MSC 068 stringer lowerback.ipt:1
- Mate:66: MSC 062 stringer back ^^.ipt:2 ↔ MSC 068 stringer lowerback.ipt:1
- Tangent:10: MSC 031 sheet lowerback.ipt:1 ↔ MSC 068 stringer lowerback.ipt:1
- [WeldJoint] (-50 mm): MSC 051 rib back.ipt:7 ↔ MSC 051 rib back.ipt:8
- [WeldJoint] (-50 mm): MSC 051 rib back.ipt:8 ↔ MSC 052 rib board.ipt:5
- [WeldJoint] (-50 mm): MSC 052 rib board.ipt:4 ↔ MSC 051 rib back.ipt:7
- [Flush]: MSC 052 rib board.ipt:5 ↔ MSC 053 rib belly.ipt:4
- [Flush]: MSC 052 rib board.ipt:5 ↔ MSC 053 rib belly.ipt:4
- [Mate]: MSC 052 rib board.ipt:5 ↔ MSC 053 rib belly.ipt:4
- [WeldJoint] (-50 mm): MSC 053 rib belly.ipt:3 ↔ MSC 053 rib belly.ipt:4
- Rigid:139 [WeldJoint] (-500 mm): MSC 051 rib back.ipt:1 ↔ MSC 051 rib back.ipt:7
- Rigid:140 [WeldJoint] (2 mm): MSC 063 stringer board #.ipt:1 ↔ MSC 063 stringer board #.ipt:4
- Rigid:141 [WeldJoint]: MSC 064 stringer board ##.ipt:1 ↔ MSC 064 stringer board ##.ipt:4
- Rigid:142 [WeldJoint]: MSC 065 stringer board ###.ipt:1 ↔ MSC 065 stringer board ###.ipt:4
- Rigid:143 [WeldJoint]: MSC 066 stringer board ####.ipt:1 ↔ MSC 066 stringer board ####.ipt:4
- Rigid:144 [WeldJoint]: MSC 067 stringer board belly.ipt:2 ↔ MSC 067 stringer board belly.ipt:8
- Rigid:145 [WeldJoint]: MSC 067 stringer board belly.ipt:1 ↔ MSC 067 stringer board belly.ipt:7
- Rigid:146 [WeldJoint]: MSC 067 stringer board belly.ipt:3 ↔ MSC 067 stringer board belly.ipt:6
- Rigid:147 [WeldJoint]: MSC 067 stringer board belly.ipt:4 ↔ MSC 067 stringer board belly.ipt:5
- Rigid:148 [WeldJoint]: MSC 063 stringer board #.ipt:2 ↔ MSC 063 stringer board #.ipt:3
- Rigid:149 [WeldJoint]: MSC 064 stringer board ##.ipt:2 ↔ MSC 064 stringer board ##.ipt:3
- Rigid:150 [WeldJoint]: MSC 065 stringer board ###.ipt:2 ↔ MSC 065 stringer board ###.ipt:3
- Rigid:151 [WeldJoint]: MSC 066 stringer board ####.ipt:2 ↔ MSC 066 stringer board ####.ipt:3
- Rigid:152 [WeldJoint]: MSC 061 stringer back ^.ipt:1 ↔ MSC 061 stringer back ^.ipt:3
- Rigid:153 [WeldJoint]: MSC 061 stringer back ^.ipt:2 ↔ MSC 061 stringer back ^.ipt:4
- Rigid:154 [WeldJoint]: MSC 062 stringer back ^^.ipt:2 ↔ MSC 062 stringer back ^^.ipt:3
- Rigid:155 [WeldJoint]: MSC 062 stringer back ^^.ipt:1 ↔ MSC 062 stringer back ^^.ipt:4
- Flush:56 (200 mm): MSC 073 ridge 3.ipt:1 ↔ MSC 027 sheet board face 1.ipt:1
- Flush:57: MSC 071 ridge 1.ipt:1 ↔ MSC 073 ridge 3.ipt:1
- Mate:68: MSC 071 ridge 1.ipt:1 ↔ MSC 073 ridge 3.ipt:1
- Flush:58 (200 mm): MSC 072 ridge 2.ipt:1
- Rotational:2 [RevoluteJoint]: ISO 5251 Bends 3D without straight ends(90 deg) DN150 11 11.ipt:1 ↔ МОО 061 труба верх 1.ipt:2
- Mate:69: MSC 027 sheet board face 1.ipt:1 ↔ MSC 075 face 2.ipt:1
- Flush:60: MSC 027 sheet board face 1.ipt:1 ↔ MSC 075 face 2.ipt:1
- Flush:61: MSC 075 face 2.ipt:1
- Rigid:156 [WeldJoint]: MSC 074 face 1.ipt:1 ↔ МОО 062 труба верх 2.ipt:1
- Rigid:157 [WeldJoint]: MSC 074 face 1.ipt:1 ↔ МОО 063 труба верх 3.ipt:1
- Mate:70: MSC 042 sheet belly-neck.ipt:1 ↔ MSC 074 face 1.ipt:1
- Flush:62: MSC 074 face 1.ipt:1
- Mate:71: MSC 042 sheet belly-neck.ipt:1 ↔ MSC 074 face 1.ipt:1
- Rigid:159 [WeldJoint] (-200 mm): MSC 074 face 1.ipt:1 ↔ МОО 061 труба верх 1.ipt:1
- Flush:76: MSC 076 face 3.ipt:1
- Mate:75: MSC 027 sheet board face 1.ipt:1 ↔ MSC 076 face 3.ipt:1
- Mate:76: MSC 075 face 2.ipt:1 ↔ MSC 076 face 3.ipt:1
- Mate:77: MSC 073 ridge 3.ipt:1 ↔ MSC 077 face 4.ipt:1
- Flush:77: MSC 077 face 4.ipt:1
- Flush:78: MSC 073 ridge 3.ipt:1 ↔ MSC 077 face 4.ipt:1
- Rigid:160 [WeldJoint]: MSC 066 stringer board ####.ipt:9 ↔ MSC 066 stringer board ####.ipt:8
- Mate:78: ASY MSC 010 cone.iam:1 ↔ MSC 021 sheet left board hip.ipt:1
- Tangent:11 (30 mm): ASY MSC 010 cone.iam:1 ↔ MSC 031 sheet lowerback.ipt:1
- Mate:79: ISO 5251 Concentric reducers DN80 x DN65 3,2 3,2.ipt:1 ↔ ASY MSC 010 cone.iam:1
- Flush:79: ASY MSC 010 cone.iam:1
- Rigid:161 [WeldJoint] (2 mm): MSC 052 rib board.ipt:1 ↔ MSC 063 stringer board #.ipt:4
- Rigid:162 [WeldJoint] (2 mm): MSC 052 rib board.ipt:1 ↔ MSC 066 stringer board ####.ipt:1
- Rigid:163 [WeldJoint] (2 mm): MSC 052 rib board.ipt:1 ↔ MSC 065 stringer board ###.ipt:1
- Rigid:164 [WeldJoint] (2 mm): MSC 052 rib board.ipt:1 ↔ MSC 064 stringer board ##.ipt:1
- Rigid:165 [WeldJoint] (-50 mm): MSC 051 rib back.ipt:3 ↔ MSC 052 rib board_CPY:2
- Mate:80: MSC 074 face 1.ipt:1 ↔ MSC 077 face 4.ipt:1
- Mate:81: MSC 073 ridge 3.ipt:1 ↔ MSC 072 ridge 2.ipt:1
- Flush:80: MSC 073 ridge 3.ipt:1 ↔ MSC 072 ridge 2.ipt:1
- Flush:81: MSC 071 ridge 1.ipt:1 ↔ MSC 072 ridge 2.ipt:1
- Rigid:166 [WeldJoint] (2 mm): MSC 065 stringer board ###.ipt:2 ↔ MSC 052 rib board.ipt:3
- Rigid:167 [WeldJoint] (2 mm): MSC 064 stringer board ##.ipt:2 ↔ MSC 052 rib board.ipt:3
- Rigid:168 [WeldJoint] (2 mm): MSC 052 rib board.ipt:3 ↔ MSC 063 stringer board #.ipt:3
- Rigid:169 [WeldJoint] (-50 mm): MSC 051 rib back.ipt:2 ↔ MSC 052 rib board_CPY:1
- Mate:82: ASY MSC 090 base frame.iam:1 ↔ ASY MSC 010 cone.iam:1
## Named parameters: Бак_нахлест_фланца = 25 mm, d230_d194 = 0 mm, d231_d195 = 0 mm, d232_d160 = 0 mm, d233_d161 = 0 mm, d322_d320 = 50 mm, d384_d346 = 0 mm, d385_d359 = -50 mm, d386_d341 = 0 mm, d387_d342 = 0 mm, d388_d243 = -50 mm, d389_d246 = -50 mm, d390_d128 = -50 mm
